# Autodesk Inventor assembly: 3000_Sample Assembly
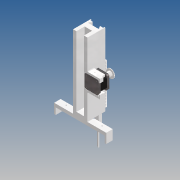
[picture p0: Inventor's stored thumbnail of the model, 180x180]
Saved by Autodesk Inventor 2020 (Build 240168000, 168)
## iProperties
Created: 2019-11-07
Part Number: 3000_Sample Assembly
Document SubType Name: Assembly
Designer: RFLab
Author: RFLab
## Documents named in this file (8)
- C:\Users\RFLab\Dropbox\MPI Group Folder\MPS\Inventor_Parts\Parts Numbered - OSMPI\3xxx_Sample Assembly\3000_Sample Assembly.iam
- C:\Users\RFLab\Dropbox\MPI Group Folder\MPS\Inventor_Parts\Parts Numbered - OSMPI\3xxx_Sample Assembly\32xx_ Motor and Driving\321x_Stepper Motor Parts\3211_Stepper Motor_V1.ipt
- C:\Users\RFLab\Dropbox\MPI Group Folder\MPS\Inventor_Parts\Parts Numbered - OSMPI\3xxx_Sample Assembly\31xx_Sample Rails\3101_Sample Rail Base_V1.ipt
- C:\Users\RFLab\Dropbox\MPI Group Folder\MPS\Inventor_Parts\Parts Numbered - OSMPI\3xxx_Sample Assembly\31xx_Sample Rails\3102_Dovetail Slider_V1.ipt
- C:\Users\RFLab\Dropbox\MPI Group Folder\MPS\Inventor_Parts\Parts Numbered - OSMPI\3xxx_Sample Assembly\31xx_Sample Rails\3103_Bulb Arm_V1.ipt
- C:\Users\RFLab\Dropbox\MPI Group Folder\MPS\Inventor_Parts\Parts Numbered - OSMPI\3xxx_Sample Assembly\32xx_ Motor and Driving\322x_Motor Mechanical Connectors\3222_Motor Rack_V1.ipt
- C:\Users\RFLab\Dropbox\MPI Group Folder\MPS\Inventor_Parts\Parts Numbered - OSMPI\3xxx_Sample Assembly\32xx_ Motor and Driving\322x_Motor Mechanical Connectors\3221_Motor Pinion_V1.ipt
- C:\Users\RFLab\Dropbox\MPI Group Folder\MPS\Inventor_Parts\Parts Numbered - OSMPI\3xxx_Sample Assembly\31xx_Sample Rails\3104_Example Bulb_V1.ipt
## Components (7 placed, 7 different names)
1. 3101_Sample Rail Base_V1:1 — Mate:1, Mate:2, Mate:13, Mate:14, Mate:15, Flush:3, Mate:16, Mate:17
2. 3102_Dovetail Slider_V1:1 — Mate:1, Mate:2, Mate:3, Mate:4, Flush:2, Mate:25, Mate:26, Mate:27
3. 3222_Motor Rack_V1:1 — Mate:3, Mate:4, Flush:2
4. 3211_Stepper Motor_V1:1 — Flush:3, Mate:16, Mate:17, Mate:21, Mate:22
5. 3221_Motor Pinion_V1:1 — Mate:21, Mate:22
6. 3104_Example Bulb_V1:1
7. 3103_Bulb Arm_V1:1 — Mate:25, Mate:26, Mate:27
## Relationships (16: Mate 14, Flush 2)
- Mate:1: 3101_Sample Rail Base_V1:1 ↔ 3102_Dovetail Slider_V1:1
- Mate:2 (-0.3 mm): 3101_Sample Rail Base_V1:1 ↔ 3102_Dovetail Slider_V1:1
- Mate:3: 3102_Dovetail Slider_V1:1 ↔ 3222_Motor Rack_V1:1
- Mate:4: 3102_Dovetail Slider_V1:1 ↔ 3222_Motor Rack_V1:1
- Flush:2: 3102_Dovetail Slider_V1:1 ↔ 3222_Motor Rack_V1:1
- Mate:13: 3101_Sample Rail Base_V1:1
- Mate:14: 3101_Sample Rail Base_V1:1
- Mate:15: 3101_Sample Rail Base_V1:1
- Flush:3: 3101_Sample Rail Base_V1:1 ↔ 3211_Stepper Motor_V1:1
- Mate:16: 3101_Sample Rail Base_V1:1 ↔ 3211_Stepper Motor_V1:1
- Mate:17: 3101_Sample Rail Base_V1:1 ↔ 3211_Stepper Motor_V1:1
- Mate:21: 3211_Stepper Motor_V1:1 ↔ 3221_Motor Pinion_V1:1
- Mate:22: 3211_Stepper Motor_V1:1 ↔ 3221_Motor Pinion_V1:1
- Mate:25: 3102_Dovetail Slider_V1:1 ↔ 3103_Bulb Arm_V1:1
- Mate:26: 3102_Dovetail Slider_V1:1 ↔ 3103_Bulb Arm_V1:1
- Mate:27: 3102_Dovetail Slider_V1:1 ↔ 3103_Bulb Arm_V1:1
